# Autodesk Inventor assembly: Assembly_MDF_Block
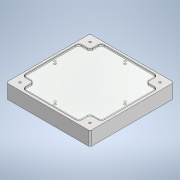
[picture p0: Inventor's stored thumbnail of the model, 180x180]
Saved by Autodesk Inventor 2021 (Build 250183000, 183)
## iProperties
Created: 2020-07-24
Part Number: Assembly_MDF_Block
Document SubType Name: Assembly
Designer: CASE-SMALL2
Author: CASE-SMALL2
## Documents named in this file (3)
- C:\Users\CASE-SMALL2\Google Drive\Unicorn 2020\CAD_V2\Manufacturing\Assembly_MDF_Block.iam
- C:\Users\CASE-SMALL2\Google Drive\Unicorn 2020\CAD_V2\Manufacturing\MDF_Block.ipt
- C:\Users\CASE-SMALL2\Google Drive\Unicorn 2020\CAD_V2\Manufacturing\AcrylicPlateForFixturePlate.ipt
## Components (2 placed, 2 different names)
1. MDF_Block:1 — Flush:1
2. AcrylicPlateForFixturePlate:1 — Flush:1
## Relationships (1: Flush 1)
- Flush:1: MDF_Block:1 ↔ AcrylicPlateForFixturePlate:1
